# Autodesk Inventor assembly: Assembly2
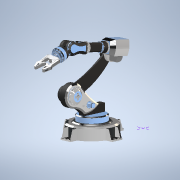
[picture p0: Inventor's stored thumbnail of the model, 180x180]
Saved by Autodesk Inventor 2022 (Build 260153000, 153)
## iProperties
Created: 2023-12-01
Part Number: Assembly2
Document SubType Name: Assembly
Designer: harshidd
Author: harshidd
## Documents named in this file (9)
- C:\Users\lando\PROJECTS\Robotic arm\robotic-arm-38.snapshot.3 (1)\Assembly2.iam
- C:\Users\lando\PROJECTS\Robotic arm\robotic-arm-38.snapshot.3 (1)\base.ipt
- C:\Users\lando\PROJECTS\Robotic arm\robotic-arm-38.snapshot.3 (1)\Part2.ipt
- C:\Users\lando\PROJECTS\Robotic arm\robotic-arm-38.snapshot.3 (1)\Part3.ipt
- C:\Users\lando\PROJECTS\Robotic arm\robotic-arm-38.snapshot.3 (1)\Part4.ipt
- C:\Users\lando\PROJECTS\Robotic arm\robotic-arm-38.snapshot.3 (1)\Part5.ipt
- C:\Users\lando\PROJECTS\Robotic arm\robotic-arm-38.snapshot.3 (1)\Part6.ipt
- C:\Users\lando\PROJECTS\Robotic arm\robotic-arm-38.snapshot.3 (1)\Part7.ipt
- C:\Users\lando\PROJECTS\Robotic arm\robotic-arm-38.snapshot.3 (1)\Part8.ipt
## Components (9 placed, 8 different names)
1. base:1 — Insert:1
2. Part2:1 — Insert:1, Insert:2
3. Part3:1 — Insert:2, Insert:3
4. Part4:1 — Insert:3, Insert:4
5. Part5:1 — Insert:4, Insert:5
6. Part6:1 — Insert:5, Insert:6
7. Part7:1 — Insert:6, Mate:1, Mate:2, Mate:3, Mate:4
8. Part8:1 — Mate:1, Mate:2
9. Part8:2 — Mate:3, Mate:4
## Relationships (10: Insert 6, Mate 4)
- Insert:1: base:1 ↔ Part2:1
- Insert:2: Part2:1 ↔ Part3:1
- Insert:3: Part3:1 ↔ Part4:1
- Insert:4: Part4:1 ↔ Part5:1
- Insert:5: Part5:1 ↔ Part6:1
- Insert:6: Part6:1 ↔ Part7:1
- Mate:1: Part7:1 ↔ Part8:1
- Mate:2: Part7:1 ↔ Part8:1
- Mate:3: Part7:1 ↔ Part8:2
- Mate:4: Part7:1 ↔ Part8:2
